# Autodesk Inventor assembly: 手動ステージ
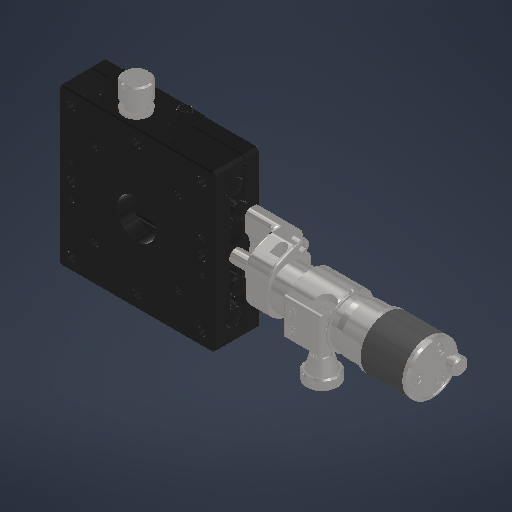
[picture p0: Inventor's stored thumbnail of the model, 512x512]
Saved by Autodesk Inventor 2026 (Build 300175050, 175E)
## iProperties
Created: 2025-07-10
Part Number: 手動ステージ
Document SubType Name: Assembly
Designer: jin20
Author: jin20
## Documents named in this file (3)
- C:\Users\jin20\Documents\装置CAD\RamanSystem\Stage\手動ステージ\手動ステージ.iam
- C:\Users\jin20\Documents\装置CAD\RamanSystem\Stage\手動ステージ\手動ステージ_02.ipt
- C:\Users\jin20\Documents\装置CAD\RamanSystem\Stage\手動ステージ\手動ステージ_01.ipt
## Components (2 placed, 2 different names)
1. 手動ステージ_02:1 — 挿入:1, 挿入:2, 挿入:3, 挿入:4
2. 手動ステージ_01:1 — 挿入:1, 挿入:2, 挿入:3, 挿入:4
## Relationships (4: Insert 4)
- 挿入:1 [Insert]: 手動ステージ_02:1 ↔ 手動ステージ_01:1
- 挿入:2 [Insert]: 手動ステージ_02:1 ↔ 手動ステージ_01:1
- 挿入:3 [Insert]: 手動ステージ_02:1 ↔ 手動ステージ_01:1
- 挿入:4 [Insert]: 手動ステージ_02:1 ↔ 手動ステージ_01:1
